# Autodesk Inventor assembly: Bat_contacts_v2_round
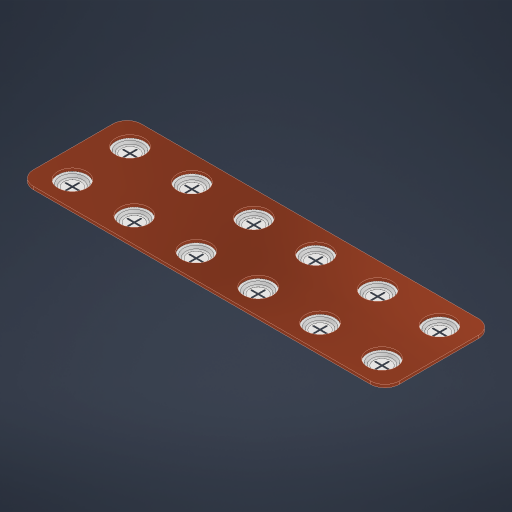
[picture p0: Inventor's stored thumbnail of the model, 512x512]
Saved by Autodesk Inventor 2024.3 (Build 283343010, 343A)
## iProperties
Created: 2025-05-14
Part Number: Bat_contacts_v2_round
Document SubType Name: Assembly
Designer: David
Author: David
## Documents named in this file (3)
- C:\Users\David\Documents\FTAG\E-16\Batterie\Batterie_Konstruktion\E-16 Batterie\Bat_contacts_v2_round.iam
- C:\Users\David\Documents\FTAG\E-16\Batterie\Batterie_Konstruktion\E-16 Batterie\bat_contacts_v2_contact_round.ipt
- C:\Users\David\Documents\FTAG\E-16\Batterie\Batterie_Konstruktion\E-16 Batterie\bat_contacts_v2_plate_hole.ipt
## Components (13 placed, 2 different names)
1. bat_contacts_v2_plate_hole:1 — Einfügen:1
2. bat_contacts_v2_contact_round:1 — Einfügen:1
3. bat_contacts_v2_contact_round:2
4. bat_contacts_v2_contact_round:3
5. bat_contacts_v2_contact_round:4
6. bat_contacts_v2_contact_round:5
7. bat_contacts_v2_contact_round:6
8. bat_contacts_v2_contact_round:7
9. bat_contacts_v2_contact_round:8
10. bat_contacts_v2_contact_round:9
11. bat_contacts_v2_contact_round:10
12. bat_contacts_v2_contact_round:11
13. bat_contacts_v2_contact_round:12
## Component patterns: (12 elements, first: bat_contacts_v2_contact_round:1)
## Relationships (1: Insert 1)
- Einfügen:1 [Insert]: bat_contacts_v2_plate_hole:1 ↔ bat_contacts_v2_contact_round:1
